# Autodesk Inventor assembly: Kamera_w_uchwycie
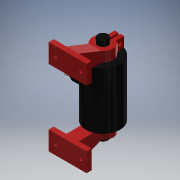
[picture p0: Inventor's stored thumbnail of the model, 180x180]
Saved by Autodesk Inventor 2017 (Build 210142000, 142)
## iProperties
Part Number: Kamera_w_uchwycie
Material: Ogólny
Document SubType Name: Assembly
Designer: Wojciech
Author: Wojciech
## Documents named in this file (3)
- C:\Users\Wojciech\Documents\Projekty\Balancer\Model 3D\Kamera_w_uchwycie.iam
- C:\Users\Wojciech\Documents\Projekty\Balancer\Model 3D\Kamera.ipt
- C:\Users\Wojciech\Documents\Projekty\Balancer\Model 3D\Kamera_uchwyt.ipt
## Components (3 placed, 2 different names)
1. Kamera:1 — Zestawiający:2, Zestawiający:3, Zestawiający:4, Zestawiający:5
2. Kamera_uchwyt:1 — Równoległy:1, Równoległy:2, Zestawiający:1, Zestawiający:2, Zestawiający:4
3. Kamera_uchwyt:2 — Równoległy:1, Równoległy:2, Zestawiający:1, Zestawiający:3, Zestawiający:5
## Relationships (7: Mate 5, Flush 2)
- Równoległy:1 [Flush]: Kamera_uchwyt:1 ↔ Kamera_uchwyt:2
- Równoległy:2 [Flush]: Kamera_uchwyt:1 ↔ Kamera_uchwyt:2
- Zestawiający:1 [Mate]: Kamera_uchwyt:1 ↔ Kamera_uchwyt:2
- Zestawiający:2 [Mate]: Kamera:1 ↔ Kamera_uchwyt:1
- Zestawiający:3 [Mate]: Kamera:1 ↔ Kamera_uchwyt:2
- Zestawiający:4 [Mate]: Kamera:1 ↔ Kamera_uchwyt:1
- Zestawiający:5 [Mate]: Kamera:1 ↔ Kamera_uchwyt:2
